# Autodesk Inventor assembly: holder_wheel_pair
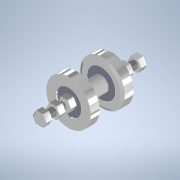
[picture p0: Inventor's stored thumbnail of the model, 180x180]
Saved by Autodesk Inventor 2020.3 (Build 243373000, 373)
## iProperties
Created: 2021-03-25
Part Number: holder_wheel_pair
Document SubType Name: Assembly
Designer: patry
Mass: 73.5609 g
Surface Area: 155.822 cm^2
Volume: 27.2448 cm^3
Density: 2.7 g/cm^3
Author: patry
## Documents named in this file (5)
- C:\Users\patry\Desktop\Semestr 7\Inzynierka\Projekt inventor\Ariadna_inzynierka\Workspaces\Obszar roboczy\Obszar roboczy\Naped\Kola\holder_wheel_pair.iam
- C:\Users\patry\Desktop\Semestr 7\Inzynierka\Projekt inventor\Ariadna_inzynierka\Workspaces\Obszar roboczy\Obszar roboczy\Naped\Sruby\M5_nut_5mm.ipt
- C:\Users\patry\Desktop\Semestr 7\Inzynierka\Projekt inventor\Ariadna_inzynierka\Workspaces\Obszar roboczy\Obszar roboczy\Naped\Kola\single_wheel_dummie.iam
- C:\Users\patry\Desktop\Semestr 7\Inzynierka\Projekt inventor\Ariadna_inzynierka\Workspaces\Obszar roboczy\Obszar roboczy\Naped\Sruby\M5_70_shaft.ipt
- C:\Users\patry\Desktop\Semestr 7\Inzynierka\Projekt inventor\Ariadna_inzynierka\Workspaces\Obszar roboczy\Obszar roboczy\Naped\Sruby\tuleja_M5_M10_15.ipt
## Components (10 placed, 4 different names)
1. M5_nut_5mm:1 — Zestawiające:17, Zestawiające:20, Zestawiające:28
2. M5_nut_5mm:5 — Zestawiające:17, Zestawiające:22, Zestawiające:27, Równoległe:1
3. single_wheel_dummie:1 [sub-assembly] — Zestawiające:20, Zestawiające:29, Zestawiające:40
4. single_wheel_dummie:2 [sub-assembly] — Zestawiające:22, Zestawiające:30
5. M5_70_shaft:1 — Zestawiające:27, Zestawiające:28, Zestawiające:29, Zestawiające:30, Równoległe:1, Zestawiające:31, Zestawiające:32, Zestawiające:33, Zestawiające:36, Zestawiające:37, Zestawiające:38, Zestawiające:39
6. M5_nut_5mm:6 — Zestawiające:31, Zestawiające:34
7. M5_nut_5mm:7 — Zestawiające:32, Zestawiające:33, Zestawiające:34
8. M5_nut_5mm:8 — Zestawiające:37, Zestawiające:38
9. M5_nut_5mm:9 — Zestawiające:36
10. tuleja_M5_M10_15:1 — Zestawiające:39, Zestawiające:40
## Relationships (18: Mate 17, Flush 1)
- Zestawiające:17 [Mate] (27 mm): M5_nut_5mm:1 ↔ M5_nut_5mm:5
- Zestawiające:20 [Mate]: M5_nut_5mm:1 ↔ single_wheel_dummie:1
- Zestawiające:22 [Mate]: M5_nut_5mm:5 ↔ single_wheel_dummie:2
- Zestawiające:27 [Mate]: M5_nut_5mm:5 ↔ M5_70_shaft:1
- Zestawiające:28 [Mate]: M5_nut_5mm:1 ↔ M5_70_shaft:1
- Zestawiające:29 [Mate]: single_wheel_dummie:1 ↔ M5_70_shaft:1
- Zestawiające:30 [Mate]: single_wheel_dummie:2 ↔ M5_70_shaft:1
- Równoległe:1 [Flush] (16.5 mm): M5_nut_5mm:5 ↔ M5_70_shaft:1
- Zestawiające:31 [Mate]: M5_70_shaft:1 ↔ M5_nut_5mm:6
- Zestawiające:32 [Mate]: M5_70_shaft:1 ↔ M5_nut_5mm:7
- Zestawiające:33 [Mate] (-5 mm): M5_70_shaft:1 ↔ M5_nut_5mm:7
- Zestawiające:34 [Mate] (5 mm): M5_nut_5mm:6 ↔ M5_nut_5mm:7
- [Mate] (5 mm): M5_nut_5mm:8 ↔ M5_nut_5mm:9
- Zestawiające:36 [Mate]: M5_70_shaft:1 ↔ M5_nut_5mm:9
- Zestawiające:37 [Mate]: M5_70_shaft:1 ↔ M5_nut_5mm:8
- Zestawiające:38 [Mate] (-5 mm): M5_70_shaft:1 ↔ M5_nut_5mm:8
- Zestawiające:39 [Mate]: M5_70_shaft:1 ↔ tuleja_M5_M10_15:1
- Zestawiające:40 [Mate]: single_wheel_dummie:1 ↔ tuleja_M5_M10_15:1
## Named parameters: d47_d46 = 5 mm
